# Autodesk Inventor assembly: 2. P+K+O+PCB
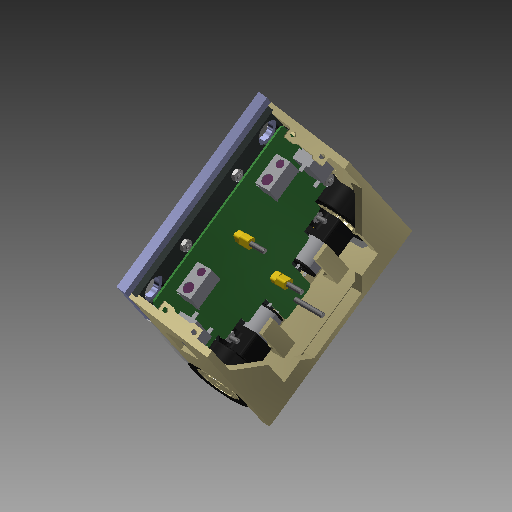
[picture p0: Inventor's stored thumbnail of the model, 512x512]
Saved by Autodesk Inventor 2017 (Build 210142000, 142)
## iProperties
Created: 2016-11-21
Part Number: 2. P+K+O+PCB
Document SubType Name: Assembly
Designer: Shichi
Author: Shichi
## Documents named in this file (6)
- E:\h3fty\H3FTY\Model\2. P+K+O+PCB.iam
- C:\Users\Shichi\Documents\Inventor\Content Center Files\R2017\en-US\AS 1112 (2)\AS 1112 - M2,5  Type 5.ipt
- E:\h3fty\H3FTY\Model\Inne\Podkladka.ipt
- E:\h3fty\H3FTY\Model\PCB\PCB+Czujniki.iam
- E:\h3fty\H3FTY\Model\1. Podstawa+Kola+Obudowa.iam
- E:\h3fty\H3FTY\Model\Inne\Podkladka_5mm.ipt
## Components (8 placed, 5 different names)
1. 1. Podstawa+Kola+Obudowa:1 [sub-assembly] — Insert:1, Insert:2
2. PCB+Czujniki:1 [sub-assembly] — Insert:1, Insert:2, Insert:3, Insert:4, Insert:5, Insert:7
3. Podkladka:1 — Insert:4, Insert:9
4. Podkladka:2 — Insert:3, Insert:8
5. AS 1112 (2) - Metric M2,5  Type 5:2 — Insert:5
6. AS 1112 (2) - Metric M2,5  Type 5:3 — Insert:7
7. Podkladka_5mm:1 — Insert:8
8. Podkladka_5mm:2 — Insert:9
## Relationships (8: Insert 8)
- Insert:1: 1. Podstawa+Kola+Obudowa:1 ↔ PCB+Czujniki:1
- Insert:2: 1. Podstawa+Kola+Obudowa:1 ↔ PCB+Czujniki:1
- Insert:3: PCB+Czujniki:1 ↔ Podkladka:2
- Insert:4: PCB+Czujniki:1 ↔ Podkladka:1
- Insert:5: PCB+Czujniki:1 ↔ AS 1112 (2) - Metric M2,5  Type 5:2
- Insert:7: PCB+Czujniki:1 ↔ AS 1112 (2) - Metric M2,5  Type 5:3
- Insert:8: Podkladka:2 ↔ Podkladka_5mm:1
- Insert:9: Podkladka:1 ↔ Podkladka_5mm:2
